# Autodesk Inventor assembly: Gearbox - 54 to 1
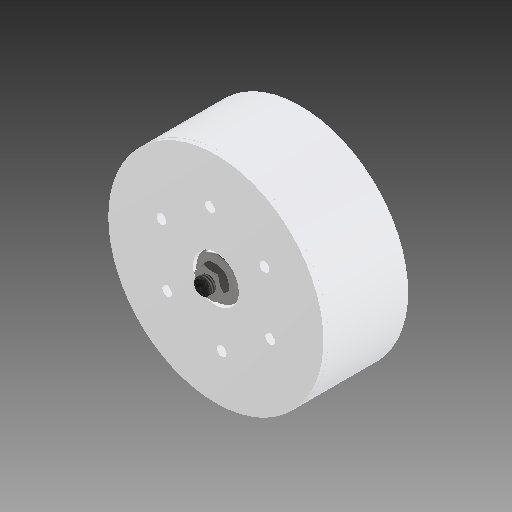
[picture p0: Inventor's stored thumbnail of the model, 512x512]
Saved by Autodesk Inventor 2017 SP1 (Build 210196100, 196)
## iProperties
Created: 2017-09-22
Part Number: Gearbox - 54 to 1
Document SubType Name: Assembly
Designer: Zach
Author: Zach
## Documents named in this file (9)
- C:\Users\Zach\Documents\GitHub\tr1\lib\Gearbox 128;1\Gearbox 128;1.iam
- C:\Users\Zach\Documents\GitHub\tr1\lib\Gearbox 128;1\Base.ipt
- C:\Users\Zach\Documents\GitHub\tr1\lib\22x8x8mm Bearing.ipt
- C:\Users\Zach\Documents\GitHub\tr1\lib\Gearbox 128;1\3mm Brass Rod.ipt
- C:\Users\Zach\Documents\Inventor\Content Center Files\R2017\en-US\ISO 4018\ISO 4018 - M8 x 50.ipt
- C:\Users\Zach\Documents\GitHub\tr1\lib\CNS 3129 - M 8 x 1.25.ipt
- C:\Users\Zach\Documents\GitHub\tr1\lib\Gearbox 128;1\GearSet 1.iam
- C:\Users\Zach\Documents\GitHub\tr1\lib\Gearbox 128;1\Cover.ipt
- C:\Users\Zach\Documents\GitHub\tr1\lib\Gearbox 128;1\Design Accelerator\Spur Gear11.ipt
## Components (19 placed, 8 different names)
1. Base:1 — Mate:1, Flush:1, Mate:4, Flush:2, Mate:5, Flush:3, Mate:6, Flush:4, Mate:7, Flush:5, Mate:8, Flush:6, Mate:9, Flush:7, Mate:161, Mate:162, Mate:163, Mate:165, Mate:167, Mate:169, Mate:172
2. Cover — Mate:155, Mate:171, Mate:172
3. ISO 4018 M8 x 50:1 — Mate:2, Mate:63, Mate:105, Mate:142, Rotation:7, Mate:155, Mate:156
4. CNS 3129 M 8:1 — Mate:105, Mate:158
5. 3mm Brass Rod:1 — Mate:4, Flush:2, Mate:168
6. 3mm Brass Rod:2 — Mate:9, Flush:7, Mate:170
7. 3mm Brass Rod:3 — Mate:8, Flush:6, Mate:159
8. 3mm Brass Rod:4 — Mate:7, Flush:5, Mate:160
9. 3mm Brass Rod:5 — Mate:6, Flush:4, Mate:164
10. 3mm Brass Rod:6 — Mate:5, Flush:3, Mate:166
11. 22x8x8mm Bearing:1 — Mate:1, Flush:1, Mate:2, Mate:63, Mate:143
12. 22x8x8mm Bearing:2 — Mate:156, Mate:158, Mate:171
13. Spur Gear1:1 — Mate:142, Mate:143, Rotation:7, Rotation:9
14. GearSet 1:1 [sub-assembly] — Mate:159, Mate:162, Rotation:8, Rotation:9
15. GearSet 1:2 [sub-assembly] — Mate:160, Mate:161, Rotation:8, Rotation:10
16. GearSet 1:3 [sub-assembly] — Mate:163, Mate:164, Rotation:10, Rotation:11
17. GearSet 1:4 [sub-assembly] — Mate:165, Mate:166, Rotation:11, Rotation:12
18. GearSet 1:5 [sub-assembly] — Mate:167, Mate:168, Rotation:12, Rotation:13
19. GearSet 1:6 [sub-assembly] — Mate:169, Mate:170, Rotation:13
## Relationships (43: Mate 29, Flush 7, RelateRotation 7)
- Mate:1: Base:1 ↔ 22x8x8mm Bearing:1
- Flush:1: Base:1 ↔ 22x8x8mm Bearing:1
- Mate:2: ISO 4018 M8 x 50:1 ↔ 22x8x8mm Bearing:1
- Mate:4: Base:1 ↔ 3mm Brass Rod:1
- Flush:2: Base:1 ↔ 3mm Brass Rod:1
- Mate:5: Base:1 ↔ 3mm Brass Rod:6
- Flush:3: Base:1 ↔ 3mm Brass Rod:6
- Mate:6: Base:1 ↔ 3mm Brass Rod:5
- Flush:4: Base:1 ↔ 3mm Brass Rod:5
- Mate:7: Base:1 ↔ 3mm Brass Rod:4
- Flush:5: Base:1 ↔ 3mm Brass Rod:4
- Mate:8: Base:1 ↔ 3mm Brass Rod:3
- Flush:6: Base:1 ↔ 3mm Brass Rod:3
- Mate:9: Base:1 ↔ 3mm Brass Rod:2
- Flush:7: Base:1 ↔ 3mm Brass Rod:2
- Mate:63: ISO 4018 M8 x 50:1 ↔ 22x8x8mm Bearing:1
- Mate:105: ISO 4018 M8 x 50:1 ↔ CNS 3129 M 8:1
- Mate:142: ISO 4018 M8 x 50:1 ↔ Spur Gear1:1
- Mate:143: 22x8x8mm Bearing:1 ↔ Spur Gear1:1
- Rotation:7 [RelateRotation] (1 ul): ISO 4018 M8 x 50:1 ↔ Spur Gear1:1
- Mate:155: Cover ↔ ISO 4018 M8 x 50:1
- Mate:156: ISO 4018 M8 x 50:1 ↔ 22x8x8mm Bearing:2
- Mate:158: CNS 3129 M 8:1 ↔ 22x8x8mm Bearing:2
- Mate:159: 3mm Brass Rod:3 ↔ GearSet 1:1
- Mate:160: 3mm Brass Rod:4 ↔ GearSet 1:2
- Mate:161: Base:1 ↔ GearSet 1:2
- Mate:162: Base:1 ↔ GearSet 1:1
- Rotation:8 [RelateRotation] (0.5 ul): GearSet 1:1 ↔ GearSet 1:2
- Rotation:9 [RelateRotation] (0.5 ul): Spur Gear1:1 ↔ GearSet 1:1
- Mate:163: Base:1 ↔ GearSet 1:3
- Mate:164: 3mm Brass Rod:5 ↔ GearSet 1:3
- Mate:165: Base:1 ↔ GearSet 1:4
- Mate:166: 3mm Brass Rod:6 ↔ GearSet 1:4
- Rotation:10 [RelateRotation] (0.5 ul): GearSet 1:2 ↔ GearSet 1:3
- Rotation:11 [RelateRotation] (0.5 ul): GearSet 1:3 ↔ GearSet 1:4
- Mate:167: Base:1 ↔ GearSet 1:5
- Mate:168: 3mm Brass Rod:1 ↔ GearSet 1:5
- Mate:169: Base:1 ↔ GearSet 1:6
- Mate:170: 3mm Brass Rod:2 ↔ GearSet 1:6
- Rotation:12 [RelateRotation] (0.5 ul): GearSet 1:4 ↔ GearSet 1:5
- Rotation:13 [RelateRotation] (0.5 ul): GearSet 1:5 ↔ GearSet 1:6
- Mate:171: Cover ↔ 22x8x8mm Bearing:2
- Mate:172: Base:1 ↔ Cover
